# Autodesk Inventor assembly: Tail
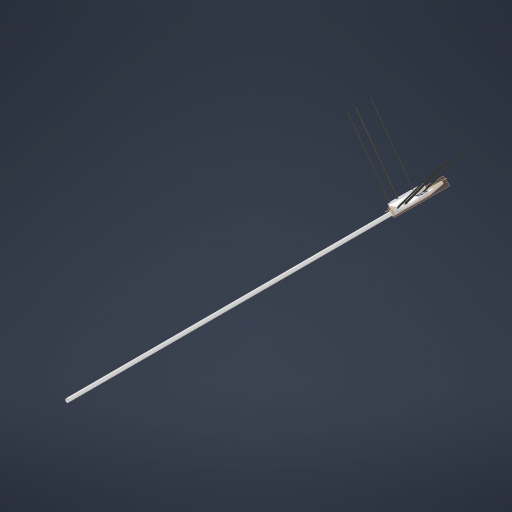
[picture p0: Inventor's stored thumbnail of the model, 512x512]
Saved by Autodesk Inventor 2023 (Build 270158000, 158)
## iProperties
Created: 2023-01-05
Part Number: Tail
Document SubType Name: Assembly
Designer: szykr
Author: szykr
## Documents named in this file (6)
- D:\Folder Instalacyjny\GitHub Pliki\Solaris\new model\Tail\Tail.iam
- D:\Folder Instalacyjny\GitHub Pliki\Solaris\new model\wingspar.ipt
- D:\Folder Instalacyjny\GitHub Pliki\Solaris\new model\Tail\Tmount.ipt
- D:\Folder Instalacyjny\GitHub Pliki\Solaris\new model\Tail\Tżebro default.ipt
- D:\Folder Instalacyjny\GitHub Pliki\Solaris\new model\Tail\Twingspar.ipt
- D:\Folder Instalacyjny\GitHub Pliki\Solaris\new model\Tail\TsmallSpar.ipt
## Components (11 placed, 5 different names)
1. wingspar:1 — Insert:1
2. Tmount:1 — Insert:1, Insert:2, Insert:3, Insert:4, Insert:5, Insert:6, Insert:8, Insert:9, Insert:10
3. Tżebro default:1 — Insert:4, Insert:5
4. Tżebro default:2 — Insert:2, Insert:3, Insert:7, Insert:12, Insert:13
5. Twingspar:1 — Insert:7
6. Twingspar:2 — Insert:6
7. Tżebro default:3 — Insert:8, Insert:9, Insert:11
8. TsmallSpar:1 — Insert:10
9. TsmallSpar:2 — Insert:11
10. TsmallSpar:3 — Insert:12
11. TsmallSpar:4 — Insert:13
## Relationships (13: Insert 13)
- Insert:1: wingspar:1 ↔ Tmount:1
- Insert:2: Tmount:1 ↔ Tżebro default:2
- Insert:3: Tmount:1 ↔ Tżebro default:2
- Insert:4: Tmount:1 ↔ Tżebro default:1
- Insert:5: Tmount:1 ↔ Tżebro default:1
- Insert:6 (-10 mm): Tmount:1 ↔ Twingspar:2
- Insert:7 (-10 mm): Tżebro default:2 ↔ Twingspar:1
- Insert:8: Tmount:1 ↔ Tżebro default:3
- Insert:9: Tmount:1 ↔ Tżebro default:3
- Insert:10 (-9.633 mm): Tmount:1 ↔ TsmallSpar:1
- Insert:11 (-9.633 mm): Tżebro default:3 ↔ TsmallSpar:2
- Insert:12 (-9.633 mm): Tżebro default:2 ↔ TsmallSpar:3
- Insert:13 (-9.633 mm): Tżebro default:2 ↔ TsmallSpar:4
## Named parameters: dlugosc = 193 mm, lotki = 4, ilosc_zeber = 6, spacing = 32.16667 mm
